# Autodesk Inventor assembly: revamped_simple_z-axis_assembly
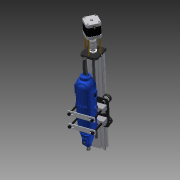
[picture p0: Inventor's stored thumbnail of the model, 180x180]
Saved by Autodesk Inventor 2014 (Build 180170000, 170)
## iProperties
Created: 2013-03-06
Part Number: revamped_simple_z-axis_assembly
Document SubType Name: Assembly
Designer: Edward
Mass: 1567.3 g
Surface Area: 2632.04 cm^2
Volume: 388.503 cm^3
Density: 4.03421 g/cm^3
Author: Edward
## Documents named in this file (28)
- C:\Users\Edward\Documents\GitHub\Shapeoko_Experimental\Shapeoko_SM\Autodesk_Inventor_Project\revamped_simple_z-axis_assembly.iam
- C:\Users\Edward\Documents\GitHub\Shapeoko_Experimental\Shapeoko_SM\Autodesk_Inventor_Project\SM-H03.ipt
- C:\Users\Edward\Documents\GitHub\Shapeoko_Experimental\Shapeoko_SM\Autodesk_Inventor_Project\SM-H04.ipt
- C:\Users\Edward\Documents\GitHub\Shapeoko_Experimental\Shapeoko_SM\Autodesk_Inventor_Project\91290A113.ipt
- C:\Users\Edward\Documents\GitHub\Shapeoko_Experimental\Shapeoko_SM\Autodesk_Inventor_Project\91166A210.ipt
- C:\Users\Edward\Documents\GitHub\Shapeoko_Experimental\Shapeoko_SM\Autodesk_Inventor_Project\HNKK55.ipt
- C:\Users\Edward\Documents\GitHub\Shapeoko_Experimental\Shapeoko_SM\Autodesk_Inventor_Project\93655A021.ipt
- C:\Users\Edward\Documents\GitHub\Shapeoko_Experimental\Shapeoko_SM\Autodesk_Inventor_Project\91239A224.ipt
- C:\Users\Edward\Documents\GitHub\Shapeoko_Experimental\Shapeoko_SM\Autodesk_Inventor_Project\SM-H12.ipt
- C:\Users\Edward\Documents\GitHub\Shapeoko_Experimental\Shapeoko_SM\Autodesk_Inventor_Project\SM-H10.ipt
- C:\Users\Edward\Documents\GitHub\Shapeoko_Experimental\Shapeoko_SM\Autodesk_Inventor_Project\z-mount_plates.ipt
- C:\Users\Edward\Documents\GitHub\Shapeoko_Experimental\Shapeoko_SM\Autodesk_Inventor_Project\z-bearing.ipt
- C:\Users\Edward\Documents\GitHub\Shapeoko_Experimental\Shapeoko_SM\Autodesk_Inventor_Project\M1173041- NEMA 17.ipt
- C:\Users\Edward\Documents\GitHub\Shapeoko_Experimental\Shapeoko_SM\Autodesk_Inventor_Project\z-axis shim.ipt
- C:\Users\Edward\Documents\GitHub\Shapeoko_Experimental\Shapeoko_SM\Autodesk_Inventor_Project\spindle_mount_plate.ipt
- C:\Users\Edward\Documents\GitHub\Shapeoko_Experimental\Shapeoko_SM\Autodesk_Inventor_Project\492-1101-ND.ipt
- C:\Users\Edward\Documents\GitHub\Shapeoko_Experimental\Shapeoko_SM\Autodesk_Inventor_Project\91239A228.ipt
- C:\Users\Edward\Documents\GitHub\Shapeoko_Experimental\Shapeoko_SM\Autodesk_Inventor_Project\SM-M08.ipt
- C:\Users\Edward\Documents\GitHub\Shapeoko_Experimental\Shapeoko_SM\Autodesk_Inventor_Project\B18033.ipt
- C:\Users\Edward\Documents\GitHub\Shapeoko_Experimental\Shapeoko_SM\Autodesk_Inventor_Project\B30037.iam
- C:\Users\Edward\Documents\GitHub\Shapeoko_Experimental\Shapeoko_SM\Autodesk_Inventor_Project\AS38-12-20.ipt
- C:\Users\Edward\Documents\GitHub\Shapeoko_Experimental\Shapeoko_SM\Autodesk_Inventor_Project\91239A236.ipt
- C:\Users\Edward\Documents\GitHub\Shapeoko_Experimental\Shapeoko_SM\Autodesk_Inventor_Project\SM-TM.ipt
- C:\Users\Edward\Documents\GitHub\Shapeoko_Experimental\Shapeoko_SM\Autodesk_Inventor_Project\SM-TM2.ipt
- C:\Users\Edward\Documents\GitHub\Shapeoko_Experimental\Shapeoko_SM\Autodesk_Inventor_Project\SM-H09.ipt
- C:\Users\Edward\Documents\GitHub\Shapeoko_Experimental\Shapeoko_SM\Autodesk_Inventor_Project\S2_MS300.ipt
- C:\Users\Edward\Documents\GitHub\Shapeoko_Experimental\Shapeoko_SM\Autodesk_Inventor_Project\S2_ZSCREW.ipt
- C:\Users\Edward\Documents\GitHub\Shapeoko_Experimental\Shapeoko_SM\Autodesk_Inventor_Project\SM-TM3.ipt
## Components (67 placed, 27 different names)
1. S2_MS300:1 — Mate:23, Mate:24, Flush:17, Insert:128, Angle:2
2. 93655A021:1 — Insert:118, Insert:119
3. 91239A224:1 — Insert:103
4. SM-H03:35 — Insert:103, Insert:104
5. HNKK55:5 — Mate:23, Mate:24, Insert:104
6. SM-H12:1 — Mate:31, Insert:127
7. z-mount_plates:1 — Mate:25, Mate:26, Mate:28, Flush:17, Insert:115, Insert:116, Insert:117, Mate:32, Flush:18
8. z-mount_plates:2 — Insert:108, Mate:28, Angle:1, Mate:30, Insert:120, Insert:125, Insert:131, Insert:132, Insert:133, Insert:139
9. z-bearing:1 — Insert:108, Mate:25, Mate:26, Insert:109, Insert:110
10. SM-H10:1 — Insert:109
11. SM-H10:2 — Insert:110
12. 91290A113:2
13. 91166A210:2 — Insert:115
14. 91290A113:3
15. 91166A210:3 — Insert:116
16. 91290A113:4
17. 91166A210:4 — Insert:117
18. 93655A021:4 — Insert:118, Angle:1, Mate:30, Insert:120
19. M1173041- NEMA 17:1 — Mate:31, Insert:119, Insert:123, Insert:124, Insert:127, Insert:177
20. 93655A021:5 — Insert:123
21. 93655A021:6 — Insert:125
22. 93655A021:7 — Insert:124
23. 93655A021:8
24. z-axis shim:1 — Insert:128, Mate:32, Insert:136, Insert:137, Flush:18
25. S2_ZSCREW:1 — Mate:33, Insert:177
26. spindle_mount_plate:1 — Insert:140, Insert:141, Insert:152, Angle:2, Mate:37, Insert:153, Insert:156, Insert:158, Insert:159, Insert:160, Insert:161, Insert:165, Insert:166, Mate:39, Insert:172, Mate:42, Flush:23, Flush:24
27. 492-1101-ND:1 — Insert:138
28. 492-1101-ND:2 — Insert:139
29. 492-1101-ND:3 — Insert:133
30. 492-1101-ND:4 — Insert:132
31. 492-1101-ND:5 — Insert:131
32. 91239A228:1
33. SM-H03:36 — Insert:136, Insert:138
34. 91239A228:2
35. SM-H03:37 — Insert:137
36. SM-M08:1 — Insert:140, Insert:141, Mate:33
37. B18033:4 — Insert:152, Mate:38
38. SM-H03:45 — Insert:156, Insert:157
39. B30037:7 [sub-assembly] — Mate:37, Insert:154, Insert:155
40. SM-H04:13 — Insert:157
41. AS38-12-20:1 — Insert:153, Insert:154
42. 91239A236:1 — Insert:155
43. SM-TM:1 — Insert:158, Insert:159, Tangent:1, Angle:3
44. SM-TM:2 — Insert:160, Insert:161, Mate:44, Flush:21, Flush:22, Insert:175, Insert:176
45. SM-H03:48 — Insert:166
46. B30037:8 [sub-assembly]
47. SM-H04:15
48. AS38-12-20:2 — Insert:165
49. 91239A236:2
50. B30037:9 [sub-assembly]
51. AS38-12-20:3 — Mate:38, Mate:39
52. 91239A236:3
53. B18033:5 — Insert:172, Mate:41
54. B30037:10 [sub-assembly]
55. AS38-12-20:4 — Mate:41, Mate:42
56. 91239A236:4
57. SM-TM3:1 — Tangent:1, Angle:3, Flush:23, Flush:24
58. SM-H09:2 — Insert:174
59. SM-H03:50 — Insert:174, Insert:176
60. SM-TM2:1 — Mate:44, Flush:21, Flush:22
61. SM-H03:49 — Insert:173, Insert:175
62. SM-H09:1 — Insert:173
63. SM-H09:3
64. SM-H03:51
65. SM-TM2:2
66. SM-H03:52
67. SM-H09:4
## Component patterns: (2 elements, first: SM-H09:2 + SM-H03:50 + SM-TM2:1 + SM-H03:49 + SM-H09:1)
## Relationships (83: Insert 57, Mate 16, Flush 6, Angle 3, Tangent 1)
- Insert:103: 91239A224:1 ↔ SM-H03:35
- Mate:23: S2_MS300:1 ↔ HNKK55:5
- Mate:24 (1 mm): S2_MS300:1 ↔ HNKK55:5
- Insert:104 (5.4163 mm): SM-H03:35 ↔ HNKK55:5
- Insert:108: z-mount_plates:2 ↔ z-bearing:1
- Mate:25: z-mount_plates:1 ↔ z-bearing:1
- Mate:26: z-mount_plates:1 ↔ z-bearing:1
- Mate:28: z-mount_plates:1 ↔ z-mount_plates:2
- Flush:17 (-5 mm): S2_MS300:1 ↔ z-mount_plates:1
- Insert:109: z-bearing:1 ↔ SM-H10:1
- Insert:110: z-bearing:1 ↔ SM-H10:2
- [Insert]: 91290A113:2 ↔ 91166A210:2
- [Insert]: 91290A113:3 ↔ 91166A210:3
- [Insert]: 91290A113:4 ↔ 91166A210:4
- Insert:115: z-mount_plates:1 ↔ 91166A210:2
- Insert:116: z-mount_plates:1 ↔ 91166A210:3
- Insert:117: z-mount_plates:1 ↔ 91166A210:4
- Insert:118: 93655A021:1 ↔ 93655A021:4
- Angle:1 (0 deg): z-mount_plates:2 ↔ 93655A021:4
- Mate:30: z-mount_plates:2 ↔ 93655A021:4
- Mate:31: SM-H12:1 ↔ M1173041- NEMA 17:1
- Insert:119: 93655A021:1 ↔ M1173041- NEMA 17:1
- Insert:120: z-mount_plates:2 ↔ 93655A021:4
- [Insert]: 93655A021:5 ↔ 93655A021:6
- [Insert]: 93655A021:7 ↔ 93655A021:8
- Insert:123: M1173041- NEMA 17:1 ↔ 93655A021:5
- Insert:124: M1173041- NEMA 17:1 ↔ 93655A021:7
- Insert:125: z-mount_plates:2 ↔ 93655A021:6
- Insert:127: SM-H12:1 ↔ M1173041- NEMA 17:1
- Insert:128: S2_MS300:1 ↔ z-axis shim:1
- Mate:32: z-mount_plates:1 ↔ z-axis shim:1
- Insert:131: z-mount_plates:2 ↔ 492-1101-ND:5
- Insert:132: z-mount_plates:2 ↔ 492-1101-ND:4
- Insert:133: z-mount_plates:2 ↔ 492-1101-ND:3
- [Insert]: 91239A228:1 ↔ SM-H03:36
- [Insert]: 91239A228:2 ↔ SM-H03:37
- Insert:136 (6.8137 mm): z-axis shim:1 ↔ SM-H03:36
- Insert:137 (6.8137 mm): z-axis shim:1 ↔ SM-H03:37
- Insert:138 (2.6568 mm): 492-1101-ND:1 ↔ SM-H03:36
- Insert:139 (-3.9853 mm): z-mount_plates:2 ↔ 492-1101-ND:2
- Insert:140: spindle_mount_plate:1 ↔ SM-M08:1
- Insert:141: spindle_mount_plate:1 ↔ SM-M08:1
- Mate:33: S2_ZSCREW:1 ↔ SM-M08:1
- Insert:152: spindle_mount_plate:1 ↔ B18033:4
- Angle:2 (0 deg): S2_MS300:1 ↔ spindle_mount_plate:1
- Mate:37: spindle_mount_plate:1 ↔ B30037:7
- Insert:153: spindle_mount_plate:1 ↔ AS38-12-20:1
- Insert:154: B30037:7 ↔ AS38-12-20:1
- Insert:155: B30037:7 ↔ 91239A236:1
- Insert:156: spindle_mount_plate:1 ↔ SM-H03:45
- Insert:157: SM-H03:45 ↔ SM-H04:13
- Insert:158: spindle_mount_plate:1 ↔ SM-TM:1
- Insert:159: spindle_mount_plate:1 ↔ SM-TM:1
- Insert:160: spindle_mount_plate:1 ↔ SM-TM:2
- Insert:161: spindle_mount_plate:1 ↔ SM-TM:2
- [Insert]: B30037:8 ↔ AS38-12-20:2
- [Insert]: B30037:8 ↔ 91239A236:2
- [Insert]: SM-H03:48 ↔ SM-H04:15
- Insert:165: spindle_mount_plate:1 ↔ AS38-12-20:2
- Insert:166: spindle_mount_plate:1 ↔ SM-H03:48
- [Insert]: B30037:9 ↔ AS38-12-20:3
- [Insert]: B30037:9 ↔ 91239A236:3
- Mate:38: B18033:4 ↔ AS38-12-20:3
- Mate:39: spindle_mount_plate:1 ↔ AS38-12-20:3
- Flush:18 (0.598 mm): z-mount_plates:1 ↔ z-axis shim:1
- [Insert]: B30037:10 ↔ AS38-12-20:4
- [Insert]: B30037:10 ↔ 91239A236:4
- [Mate]: B18033:5 ↔ AS38-12-20:4
- Insert:172: spindle_mount_plate:1 ↔ B18033:5
- Mate:41: B18033:5 ↔ AS38-12-20:4
- Mate:42: spindle_mount_plate:1 ↔ AS38-12-20:4
- Mate:44 (43 mm): SM-TM:2 ↔ SM-TM2:1
- Flush:21: SM-TM:2 ↔ SM-TM2:1
- Flush:22: SM-TM:2 ↔ SM-TM2:1
- Insert:173: SM-H03:49 ↔ SM-H09:1
- Insert:174: SM-H09:2 ↔ SM-H03:50
- Insert:175 (45 mm): SM-TM:2 ↔ SM-H03:49
- Insert:176 (45 mm): SM-TM:2 ↔ SM-H03:50
- Insert:177: M1173041- NEMA 17:1 ↔ S2_ZSCREW:1
- Tangent:1: SM-TM:1 ↔ SM-TM3:1
- Angle:3 (0 deg): SM-TM:1 ↔ SM-TM3:1
- Flush:23 (-60 mm): spindle_mount_plate:1 ↔ SM-TM3:1
- Flush:24 (38 mm): spindle_mount_plate:1 ↔ SM-TM3:1
## Named parameters: d159_d104 = 0 mm, d182_d39 = 0 mm, d184_d182_d39 = 0 mm, d185_d182_d39 = 0 mm, d197_d190 = 0 mm, d198_d190 = 0 mm, d101_d55_d51 = 0 mm, d212_d101_d55_d51 = 0 mm, d254_d246 = 0 mm, d255_d247 = 0 mm, d256_d249 = 0 mm, d259_d246 = 0 mm, d260_d247 = 0 mm, d267_d259_d246 = 0 mm, d268_d260_d247 = 0 mm, d269_d262 = 0 mm
